# Autodesk Inventor assembly: Assembly1
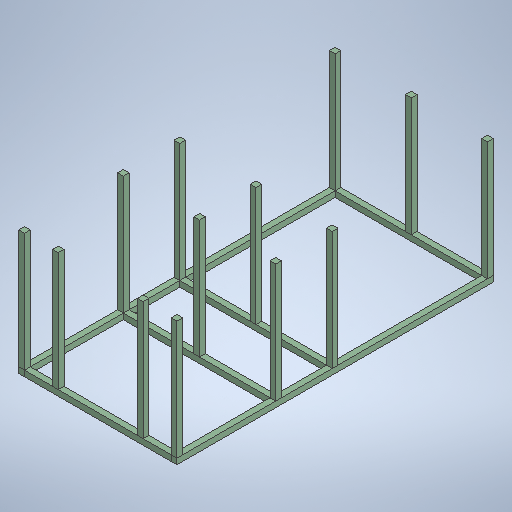
[picture p0: Inventor's stored thumbnail of the model, 512x512]
Saved by Autodesk Inventor 2025.1 (Build 291241020, 241B)
## iProperties
Created: 2024-09-16
Part Number: Assembly1
Document SubType Name: Assembly
Designer: User
Author: User
## Documents named in this file (12)
- C:\Users\User\Documents\Tburn24\Assembly1.iam
- C:\Users\User\Documents\Tburn24\16'x4x4.ipt
- C:\Users\User\Documents\Tburn24\7'5x4x4.ipt
- C:\Users\User\Documents\Tburn24\6'x4x4.ipt
- C:\Users\User\Documents\Tburn24\6'x2x4.ipt
- C:\Users\User\Documents\Tburn24\16'x2x4.ipt
- C:\Users\User\Documents\Tburn24\7'5x2x4.ipt
- C:\Users\User\Documents\Tburn24\Part11.ipt
- C:\Users\User\Documents\Tburn24\side1.ipt
- C:\Users\User\Documents\Tburn24\side2.ipt
- C:\Users\User\Documents\Tburn24\side3.ipt
- C:\Users\User\Documents\Tburn24\fside1.ipt
## Components (40 placed, 11 different names)
1. 16'x4x4:1 — Mate:1, Flush:1, Flush:2, Mate:3, Flush:5, Flush:6, Flush:7, Flush:8, Flush:9, Mate:8, Mate:9, Mate:10, Mate:11, Mate:12, Mate:13, Mate:16, Flush:12, Flush:13, Flush:14, Flush:17, Flush:20, Mate:20, Flush:34
2. 16'x4x4:2 — Mate:1, Flush:1, Flush:2, Flush:3, Mate:2, Flush:4, Mate:4, Mate:5, Mate:7, Flush:10, Flush:11, Mate:15, Mate:17, Mate:18, Flush:19, Flush:23, Flush:24, Flush:35, Mate:22, Mate:54
3. 7'5x4x4:1 — Flush:3, Mate:2, Flush:4, Mate:6, Flush:58, Flush:61
4. 7'5x4x4:2 — Mate:3, Flush:5, Flush:6, Flush:21, Flush:22, Flush:27, Mate:41
5. 7'5x4x4:3 — Flush:7, Mate:4, Flush:8, Flush:15, Flush:25, Flush:31
6. 7'5x4x4:4 — Flush:9, Mate:5, Mate:6, Mate:14, Flush:16, Flush:18, Flush:29
7. 6'x4x4:1 — Mate:7, Flush:10, Flush:11, Mate:24, Flush:36, Flush:37, Mate:59
8. 6'x4x4:1 — Mate:8, Flush:12, Flush:13, Mate:55, Mate:25, Flush:59, Mate:60, Flush:60
9. 6'x4x4:2 — Mate:9, Flush:14, Flush:15, Flush:30
10. 6'x4x4:3 — Mate:11, Mate:55
11. 6'x4x4:4 — Mate:10, Flush:24, Flush:25
12. 6'x4x4:5 — Mate:14, Flush:28, Flush:29, Mate:28, Flush:44, Mate:37, Mate:43, Flush:49
13. 6'x4x4:6 — Mate:15, Flush:26, Flush:27, Mate:29, Flush:42, Mate:39, Mate:42, Flush:48
14. 6'x4x4:7 — Mate:16, Flush:20, Flush:21, Mate:21, Flush:38, Flush:39, Flush:51
15. 6'x4x4:8 — Mate:18, Flush:18, Flush:19, Flush:28, Flush:54, Flush:55, Flush:56
16. 6'x4x4:9 — Mate:17, Flush:22, Flush:23, Flush:26, Mate:23
17. 6'x4x4:10 — Mate:13, Flush:30, Flush:31, Mate:27, Flush:43, Mate:36, Flush:45, Mate:44, Flush:50
18. 6'x4x4:23 — Flush:58, Mate:58, Mate:59
19. 6'x4x4:11 — Mate:12, Flush:16, Flush:17, Mate:50, Flush:53
20. 6'x2x4:1 — Mate:20, Flush:34, Mate:21
21. 6'x2x4:2 — Flush:35, Mate:22, Mate:23, Mate:53
22. 16'x2x4:1 — Mate:24, Flush:36, Flush:37, Mate:26, Flush:40, Flush:41, Mate:31, Symmetry:1, Mate:51, Mate:52
23. 16'x2x4:2 — Mate:25, Flush:38, Flush:39, Mate:30, Mate:32, Symmetry:1, Mate:49
24. 7'5x2x4:1 — Mate:26, Flush:40, Flush:41, Mate:58
25. 7'5x2x4:2 — Mate:27, Mate:32, Flush:43, Flush:46, Mate:47
26. 7'5x2x4:3 — Mate:28, Mate:31, Flush:44, Flush:47, Mate:38, Mate:46
27. 7'5x2x4:4 — Mate:29, Flush:42, Mate:30, Mate:40, Mate:45
28. Part11:3 — Mate:39, Mate:40, Mate:41
29. Part11:4 — Flush:47, Mate:37, Mate:38
30. Part11:5 — Mate:36, Flush:45, Flush:46
31. Part11:6 — Mate:42, Flush:48, Mate:45
32. Part11:7 — Mate:44, Flush:50, Mate:47
33. Part11:8 — Mate:43, Flush:49, Mate:46
34. side1:1 — Flush:51
35. side2:2 — Mate:49, Mate:50, Flush:53
36. side2:3 — Mate:51, Flush:54, Flush:55
37. side1:2 — Mate:52, Mate:53, Mate:54
38. side3:1 — Flush:56
39. fside1:1 — Flush:59
40. fside1:2 — Mate:60, Flush:60, Flush:61
## Relationships (111: Flush 57, Mate 53, Symmetry 1)
- Mate:1 (2260.6 mm): 16'x4x4:1 ↔ 16'x4x4:2
- Flush:1: 16'x4x4:1 ↔ 16'x4x4:2
- Flush:2: 16'x4x4:1 ↔ 16'x4x4:2
- Flush:3: 16'x4x4:2 ↔ 7'5x4x4:1
- Mate:2: 16'x4x4:2 ↔ 7'5x4x4:1
- Flush:4: 16'x4x4:2 ↔ 7'5x4x4:1
- Mate:3: 16'x4x4:1 ↔ 7'5x4x4:2
- Flush:5: 16'x4x4:1 ↔ 7'5x4x4:2
- Flush:6: 16'x4x4:1 ↔ 7'5x4x4:2
- Flush:7 (1524 mm): 16'x4x4:1 ↔ 7'5x4x4:3
- Mate:4: 16'x4x4:2 ↔ 7'5x4x4:3
- Flush:8: 16'x4x4:1 ↔ 7'5x4x4:3
- Flush:9: 16'x4x4:1 ↔ 7'5x4x4:4
- Mate:5: 16'x4x4:2 ↔ 7'5x4x4:4
- Mate:6 (2393.95 mm): 7'5x4x4:1 ↔ 7'5x4x4:4
- Mate:7: 16'x4x4:2 ↔ 6'x4x4:1
- Flush:10: 16'x4x4:2 ↔ 6'x4x4:1
- Flush:11: 16'x4x4:2 ↔ 6'x4x4:1
- Mate:8: 16'x4x4:1 ↔ 6'x4x4:1
- Mate:9: 16'x4x4:1 ↔ 6'x4x4:2
- Mate:10: 16'x4x4:1 ↔ 6'x4x4:4
- Mate:11: 16'x4x4:1 ↔ 6'x4x4:3
- Mate:12: 16'x4x4:1 ↔ 6'x4x4:11
- Mate:13: 16'x4x4:1 ↔ 6'x4x4:10
- Mate:14: 7'5x4x4:4 ↔ 6'x4x4:5
- Mate:15: 16'x4x4:2 ↔ 6'x4x4:6
- Mate:16: 16'x4x4:1 ↔ 6'x4x4:7
- Mate:17: 16'x4x4:2 ↔ 6'x4x4:9
- Mate:18: 16'x4x4:2 ↔ 6'x4x4:8
- Flush:12: 16'x4x4:1 ↔ 6'x4x4:1
- Flush:13: 16'x4x4:1 ↔ 6'x4x4:1
- Flush:14: 16'x4x4:1 ↔ 6'x4x4:2
- Flush:15: 7'5x4x4:3 ↔ 6'x4x4:2
- Flush:16: 7'5x4x4:4 ↔ 6'x4x4:11
- Flush:17: 16'x4x4:1 ↔ 6'x4x4:11
- Flush:18: 7'5x4x4:4 ↔ 6'x4x4:8
- Flush:19: 16'x4x4:2 ↔ 6'x4x4:8
- Flush:20: 16'x4x4:1 ↔ 6'x4x4:7
- Flush:21: 7'5x4x4:2 ↔ 6'x4x4:7
- Flush:22: 7'5x4x4:2 ↔ 6'x4x4:9
- Flush:23: 16'x4x4:2 ↔ 6'x4x4:9
- Flush:24: 16'x4x4:2 ↔ 6'x4x4:4
- Flush:25: 7'5x4x4:3 ↔ 6'x4x4:4
- Flush:26 (-1174.75 mm): 6'x4x4:6 ↔ 6'x4x4:9
- Flush:27: 7'5x4x4:2 ↔ 6'x4x4:6
- Flush:28 (1174.75 mm): 6'x4x4:5 ↔ 6'x4x4:8
- Flush:29: 7'5x4x4:4 ↔ 6'x4x4:5
- Flush:30 (1174.75 mm): 6'x4x4:2 ↔ 6'x4x4:10
- Flush:31: 7'5x4x4:3 ↔ 6'x4x4:10
- Mate:55 (-609.6 mm): 6'x4x4:1 ↔ 6'x4x4:3
- Mate:20: 16'x4x4:1 ↔ 6'x2x4:1
- Flush:34: 16'x4x4:1 ↔ 6'x2x4:1
- Mate:21 (-1238.25 mm): 6'x4x4:7 ↔ 6'x2x4:1
- Flush:35: 16'x4x4:2 ↔ 6'x2x4:2
- Mate:22: 16'x4x4:2 ↔ 6'x2x4:2
- Mate:23 (-1238.25 mm): 6'x4x4:9 ↔ 6'x2x4:2
- Mate:24: 6'x4x4:1 ↔ 16'x2x4:1
- Flush:36: 6'x4x4:1 ↔ 16'x2x4:1
- Flush:37: 6'x4x4:1 ↔ 16'x2x4:1
- Mate:25: 6'x4x4:1 ↔ 16'x2x4:2
- Flush:38: 6'x4x4:7 ↔ 16'x2x4:2
- Flush:39: 6'x4x4:7 ↔ 16'x2x4:2
- Mate:26: 16'x2x4:1 ↔ 7'5x2x4:1
- Flush:40: 16'x2x4:1 ↔ 7'5x2x4:1
- Flush:41: 16'x2x4:1 ↔ 7'5x2x4:1
- Mate:27: 6'x4x4:10 ↔ 7'5x2x4:2
- Mate:28: 6'x4x4:5 ↔ 7'5x2x4:3
- Mate:29: 6'x4x4:6 ↔ 7'5x2x4:4
- Flush:42: 6'x4x4:6 ↔ 7'5x2x4:4
- Mate:30: 16'x2x4:2 ↔ 7'5x2x4:4
- Mate:31: 16'x2x4:1 ↔ 7'5x2x4:3
- Mate:32: 16'x2x4:2 ↔ 7'5x2x4:2
- Flush:43: 6'x4x4:10 ↔ 7'5x2x4:2
- Flush:44: 6'x4x4:5 ↔ 7'5x2x4:3
- Symmetry:1: 16'x2x4:1 ↔ 16'x2x4:2
- Mate:36: 6'x4x4:10 ↔ Part11:5
- Flush:45: 6'x4x4:10 ↔ Part11:5
- Flush:46: 7'5x2x4:2 ↔ Part11:5
- Flush:47: 7'5x2x4:3 ↔ Part11:4
- Mate:37: 6'x4x4:5 ↔ Part11:4
- Mate:38: 7'5x2x4:3 ↔ Part11:4
- Mate:39: 6'x4x4:6 ↔ Part11:3
- Mate:40: 7'5x2x4:4 ↔ Part11:3
- Mate:41: 7'5x4x4:2 ↔ Part11:3
- Mate:42: 6'x4x4:6 ↔ Part11:6
- Mate:43: 6'x4x4:5 ↔ Part11:8
- Mate:44: 6'x4x4:10 ↔ Part11:7
- Flush:48: 6'x4x4:6 ↔ Part11:6
- Flush:49: 6'x4x4:5 ↔ Part11:8
- Flush:50: 6'x4x4:10 ↔ Part11:7
- Mate:45: 7'5x2x4:4 ↔ Part11:6
- Mate:46: 7'5x2x4:3 ↔ Part11:8
- Mate:47: 7'5x2x4:2 ↔ Part11:7
- Flush:51: 6'x4x4:7 ↔ side1:1
- Mate:49: 16'x2x4:2 ↔ side2:2
- Mate:50: 6'x4x4:11 ↔ side2:2
- Flush:53: 6'x4x4:11 ↔ side2:2
- Mate:51: 16'x2x4:1 ↔ side2:3
- Flush:54: 6'x4x4:8 ↔ side2:3
- Flush:55: 6'x4x4:8 ↔ side2:3
- Mate:52: 16'x2x4:1 ↔ side1:2
- Mate:53: 6'x2x4:2 ↔ side1:2
- Mate:54: 16'x4x4:2 ↔ side1:2
- Flush:56: 6'x4x4:8 ↔ side3:1
- Flush:58: 7'5x4x4:1 ↔ 6'x4x4:23
- Mate:58: 6'x4x4:23 ↔ 7'5x2x4:1
- Mate:59 (-609.6 mm): 6'x4x4:1 ↔ 6'x4x4:23
- Flush:59: 6'x4x4:1 ↔ fside1:1
- Mate:60: 6'x4x4:1 ↔ fside1:2
- Flush:60: 6'x4x4:1 ↔ fside1:2
- Flush:61: 7'5x4x4:1 ↔ fside1:2
